# Autodesk Inventor assembly: InteriorElectronics
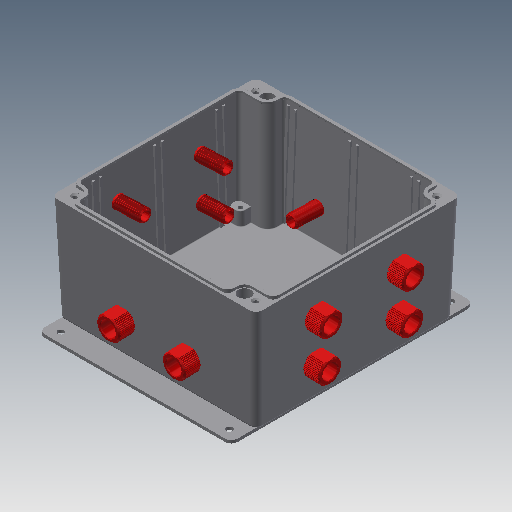
[picture p0: Inventor's stored thumbnail of the model, 512x512]
Saved by Autodesk Inventor 2018 (Build 220112000, 112)
## iProperties
Created: 2019-03-26
Part Number: InteriorElectronics
Document SubType Name: Assembly
Designer: anirudh
Author: anirudh
## Documents named in this file (4)
- D:\Silicon Sharks\2019-2020\ElectronicsHousing\Prototype3\mainEnclosure.iam
- C:\Users\anirudh\Documents\MARS Fund\MATE Robotics\Silicon Sharks\2018-2019\ElectronicsHousing\Prototype2\HousingReference(2).ipt
- C:\Users\anirudh\Documents\MARS Fund\MATE Robotics\Silicon Sharks\2018-2019\ElectronicsHousing\Prototype2\6MMPenetrator(2).ipt
- C:\Users\anirudh\Documents\MARS Fund\MATE Robotics\Silicon Sharks\2018-2019\ElectronicsHousing\Prototype2\6mmPenetratorORing(2).ipt
## Components (25 placed, 3 different names)
1. HousingReference(2):1 — Mate:26, Mate:27, Mate:28, Mate:29, Mate:30, Mate:31, Mate:32, Mate:33, Mate:34, Mate:35, Mate:36, Mate:37, Mate:38, Mate:39, Mate:40, Mate:41, Mate:42, Mate:43, Mate:44, Mate:45, Mate:46, Mate:47, Mate:48, Mate:49
2. 6MMPenetrator(2):1 — Mate:2, Mate:3, Mate:28, Mate:29
3. 6mmPenetratorORing(2):1 — Mate:2, Mate:3
4. 6MMPenetrator(2):2 — Mate:4, Mate:5, Mate:26, Mate:27
5. 6mmPenetratorORing(2):2 — Mate:4, Mate:5
6. 6MMPenetrator(2):3 — Mate:8, Mate:9, Mate:34, Mate:36
7. 6mmPenetratorORing(2):3 — Mate:8, Mate:9
8. 6MMPenetrator(2):4 — Mate:6, Mate:7, Mate:35, Mate:37
9. 6mmPenetratorORing(2):4 — Mate:6, Mate:7
10. 6MMPenetrator(2):5 — Mate:12, Mate:13, Mate:38, Mate:39
11. 6mmPenetratorORing(2):5 — Mate:12, Mate:13
12. 6MMPenetrator(2):6 — Mate:10, Mate:11, Mate:40, Mate:41
13. 6mmPenetratorORing(2):6 — Mate:10, Mate:11
14. 6MMPenetrator(2):7 — Mate:16, Mate:17, Mate:32, Mate:33
15. 6mmPenetratorORing(2):7 — Mate:16, Mate:17
16. 6MMPenetrator(2):8 — Mate:14, Mate:15, Mate:30, Mate:31
17. 6mmPenetratorORing(2):8 — Mate:14, Mate:15
18. 6MMPenetrator(2):9 — Mate:20, Mate:21, Mate:48, Mate:49
19. 6mmPenetratorORing(2):9 — Mate:20, Mate:21
20. 6MMPenetrator(2):10 — Mate:18, Mate:19, Mate:46, Mate:47
21. 6mmPenetratorORing(2):10 — Mate:18, Mate:19
22. 6MMPenetrator(2):11 — Mate:24, Mate:25, Mate:44, Mate:45
23. 6mmPenetratorORing(2):11 — Mate:24, Mate:25
24. 6MMPenetrator(2):12 — Mate:22, Mate:23, Mate:42, Mate:43
25. 6mmPenetratorORing(2):12 — Mate:22, Mate:23
## Relationships (48: Mate 48)
- Mate:2: 6MMPenetrator(2):1 ↔ 6mmPenetratorORing(2):1
- Mate:3: 6MMPenetrator(2):1 ↔ 6mmPenetratorORing(2):1
- Mate:4: 6MMPenetrator(2):2 ↔ 6mmPenetratorORing(2):2
- Mate:5: 6MMPenetrator(2):2 ↔ 6mmPenetratorORing(2):2
- Mate:6: 6MMPenetrator(2):4 ↔ 6mmPenetratorORing(2):4
- Mate:7: 6MMPenetrator(2):4 ↔ 6mmPenetratorORing(2):4
- Mate:8: 6MMPenetrator(2):3 ↔ 6mmPenetratorORing(2):3
- Mate:9: 6MMPenetrator(2):3 ↔ 6mmPenetratorORing(2):3
- Mate:10: 6MMPenetrator(2):6 ↔ 6mmPenetratorORing(2):6
- Mate:11: 6MMPenetrator(2):6 ↔ 6mmPenetratorORing(2):6
- Mate:12: 6MMPenetrator(2):5 ↔ 6mmPenetratorORing(2):5
- Mate:13: 6MMPenetrator(2):5 ↔ 6mmPenetratorORing(2):5
- Mate:14: 6MMPenetrator(2):8 ↔ 6mmPenetratorORing(2):8
- Mate:15: 6MMPenetrator(2):8 ↔ 6mmPenetratorORing(2):8
- Mate:16: 6MMPenetrator(2):7 ↔ 6mmPenetratorORing(2):7
- Mate:17: 6MMPenetrator(2):7 ↔ 6mmPenetratorORing(2):7
- Mate:18: 6MMPenetrator(2):10 ↔ 6mmPenetratorORing(2):10
- Mate:19: 6MMPenetrator(2):10 ↔ 6mmPenetratorORing(2):10
- Mate:20: 6MMPenetrator(2):9 ↔ 6mmPenetratorORing(2):9
- Mate:21: 6MMPenetrator(2):9 ↔ 6mmPenetratorORing(2):9
- Mate:22: 6MMPenetrator(2):12 ↔ 6mmPenetratorORing(2):12
- Mate:23: 6MMPenetrator(2):12 ↔ 6mmPenetratorORing(2):12
- Mate:24: 6MMPenetrator(2):11 ↔ 6mmPenetratorORing(2):11
- Mate:25: 6MMPenetrator(2):11 ↔ 6mmPenetratorORing(2):11
- Mate:26: HousingReference(2):1 ↔ 6MMPenetrator(2):2
- Mate:27: HousingReference(2):1 ↔ 6MMPenetrator(2):2
- Mate:28: HousingReference(2):1 ↔ 6MMPenetrator(2):1
- Mate:29: HousingReference(2):1 ↔ 6MMPenetrator(2):1
- Mate:30: HousingReference(2):1 ↔ 6MMPenetrator(2):8
- Mate:31: HousingReference(2):1 ↔ 6MMPenetrator(2):8
- Mate:32: HousingReference(2):1 ↔ 6MMPenetrator(2):7
- Mate:33: HousingReference(2):1 ↔ 6MMPenetrator(2):7
- Mate:34: HousingReference(2):1 ↔ 6MMPenetrator(2):3
- Mate:35: HousingReference(2):1 ↔ 6MMPenetrator(2):4
- Mate:36: HousingReference(2):1 ↔ 6MMPenetrator(2):3
- Mate:37: HousingReference(2):1 ↔ 6MMPenetrator(2):4
- Mate:38: HousingReference(2):1 ↔ 6MMPenetrator(2):5
- Mate:39: HousingReference(2):1 ↔ 6MMPenetrator(2):5
- Mate:40: HousingReference(2):1 ↔ 6MMPenetrator(2):6
- Mate:41: HousingReference(2):1 ↔ 6MMPenetrator(2):6
- Mate:42: HousingReference(2):1 ↔ 6MMPenetrator(2):12
- Mate:43: HousingReference(2):1 ↔ 6MMPenetrator(2):12
- Mate:44: HousingReference(2):1 ↔ 6MMPenetrator(2):11
- Mate:45: HousingReference(2):1 ↔ 6MMPenetrator(2):11
- Mate:46: HousingReference(2):1 ↔ 6MMPenetrator(2):10
- Mate:47: HousingReference(2):1 ↔ 6MMPenetrator(2):10
- Mate:48: HousingReference(2):1 ↔ 6MMPenetrator(2):9
- Mate:49: HousingReference(2):1 ↔ 6MMPenetrator(2):9
